# Autodesk Inventor assembly: CE-7.1.1_CE-2.1.4_LA1
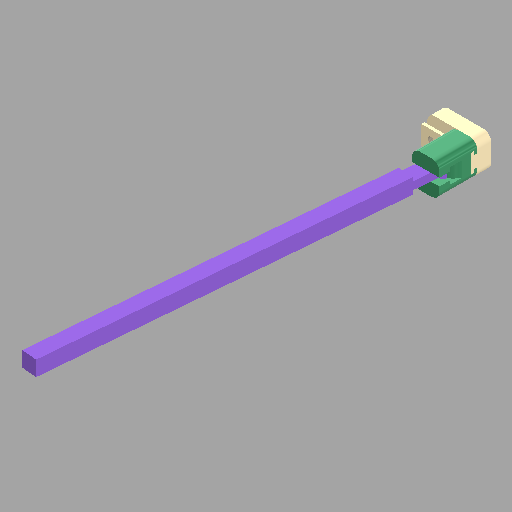
[picture p0: Inventor's stored thumbnail of the model, 512x512]
Saved by Autodesk Inventor 2024 (Build 280153000, 153)
## iProperties
Created: 2024-02-25
Part Number: CE-7.1.1_CE-2.1.4_LA1
Document SubType Name: Assembly
Designer: Alex
Author: Alex
## Documents named in this file (4)
- C:\Shared\alex-bartella-schoolwork\4z03\Week 6\Lifters\DME_Flat Core Blades 1\CE-7.1.1_CE-2.1.4_LA1.iam
- C:\Shared\alex-bartella-schoolwork\4z03\Week 6\Lifters\DME_Flat Core Blades 1\CE-7.1.1_CE-2.1.4_LA1_ULG.ipt
- C:\Shared\alex-bartella-schoolwork\4z03\Week 6\Lifters\DME_Flat Core Blades 1\CE-7.1.1_CE-2.1.4_LA1_ULC.ipt
- C:\Shared\alex-bartella-schoolwork\4z03\Week 6\Lifters\DME_Flat Core Blades 1\CE-7.1.1_CE-2.1.4_LA1_ULB_Flat.ipt
## Components (3 placed, 3 different names)
1. CE-7.1.1_CE-2.1.4_LA1_ULG:1 — Flush:1, Flush:2, Mate:1, Flush:3, Flush:4, Flush:5, Mate:2
2. CE-7.1.1_CE-2.1.4_LA1_ULC:1 — Flush:3, Flush:4, Flush:5, Mate:3, Angle:1
3. CE-7.1.1_CE-2.1.4_LA1_ULB_Flat:1 — Mate:2, Mate:3, Angle:1
## Relationships (9: Flush 5, Mate 3, Angle 1)
- Flush:1: CE-7.1.1_CE-2.1.4_LA1_ULG:1
- Flush:2: CE-7.1.1_CE-2.1.4_LA1_ULG:1
- Mate:1: CE-7.1.1_CE-2.1.4_LA1_ULG:1
- Flush:3: CE-7.1.1_CE-2.1.4_LA1_ULG:1 ↔ CE-7.1.1_CE-2.1.4_LA1_ULC:1
- Flush:4: CE-7.1.1_CE-2.1.4_LA1_ULG:1 ↔ CE-7.1.1_CE-2.1.4_LA1_ULC:1
- Flush:5: CE-7.1.1_CE-2.1.4_LA1_ULG:1 ↔ CE-7.1.1_CE-2.1.4_LA1_ULC:1
- Mate:2: CE-7.1.1_CE-2.1.4_LA1_ULG:1 ↔ CE-7.1.1_CE-2.1.4_LA1_ULB_Flat:1
- Mate:3: CE-7.1.1_CE-2.1.4_LA1_ULC:1 ↔ CE-7.1.1_CE-2.1.4_LA1_ULB_Flat:1
- Angle:1 (-5 deg): CE-7.1.1_CE-2.1.4_LA1_ULC:1 ↔ CE-7.1.1_CE-2.1.4_LA1_ULB_Flat:1
